# Autodesk Inventor assembly: Disco
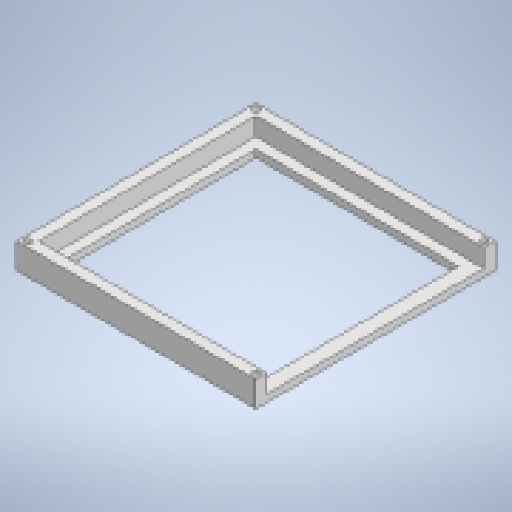
[picture p0: Inventor's stored thumbnail of the model, 512x512]
Saved by Autodesk Inventor 2024 (Build 280153000, 153)
## iProperties
Created: 2025-02-27
Part Number: Disco
Document SubType Name: Assembly
Designer: sergi
Author: sergi
## Documents named in this file (3)
- C:\Users\sergi\OneDrive\Escritorio\Projects\16. Protection catapult\Inventor\Disco.iam
- C:\Users\sergi\OneDrive\Escritorio\Projects\16. Protection catapult\Inventor\Disco_inferior.ipt
- C:\Users\sergi\OneDrive\Escritorio\Projects\16. Protection catapult\Inventor\Disco_Superior.ipt
## Components (2 placed, 2 different names)
1. Disco_inferior:1 — Nivelación:1
2. Disco_Superior:1 — Nivelación:1
## Relationships (1: Flush 1)
- Nivelación:1 [Flush]: Disco_inferior:1 ↔ Disco_Superior:1
